# Autodesk Inventor assembly: SAR330
(part 2 of 2)
- to_ball3_2_Z@1 <-> to_rail_Z@57 [Mate]: SAR330-30_r:1 ↔ SAR3_ba:54
- to_ball3_2_YZ@1 <-> to_rail_YZ@57 [Angle] (0 deg): SAR330-30_r:1 ↔ SAR3_ba:54
- to_ball3_3_XY@1 <-> to_rail_XY@58 [Mate]: SAR330-30_r:1 ↔ SAR3_ba:55
- to_ball3_3_Z@1 <-> to_rail_Z@58 [Mate]: SAR330-30_r:1 ↔ SAR3_ba:55
- to_ball3_3_YZ@1 <-> to_rail_YZ@58 [Angle] (0 deg): SAR330-30_r:1 ↔ SAR3_ba:55
- to_ball3_4_XY@1 <-> to_rail_XY@59 [Mate]: SAR330-30_r:1 ↔ SAR3_ba:56
- to_ball3_4_Z@1 <-> to_rail_Z@59 [Mate]: SAR330-30_r:1 ↔ SAR3_ba:56
- to_ball3_4_YZ@1 <-> to_rail_YZ@59 [Angle] (0 deg): SAR330-30_r:1 ↔ SAR3_ba:56
- to_ball3_5_XY@1 <-> to_rail_XY@60 [Mate]: SAR330-30_r:1 ↔ SAR3_ba:57
- to_ball3_5_Z@1 <-> to_rail_Z@60 [Mate]: SAR330-30_r:1 ↔ SAR3_ba:57
- to_ball3_5_YZ@1 <-> to_rail_YZ@60 [Angle] (0 deg): SAR330-30_r:1 ↔ SAR3_ba:57
- to_ball3_6_XY@1 <-> to_rail_XY@61 [Mate]: SAR330-30_r:1 ↔ SAR3_ba:58
- to_ball3_6_Z@1 <-> to_rail_Z@61 [Mate]: SAR330-30_r:1 ↔ SAR3_ba:58
- to_ball3_6_YZ@1 <-> to_rail_YZ@61 [Angle] (0 deg): SAR330-30_r:1 ↔ SAR3_ba:58
- to_ball3_7_XY@1 <-> to_rail_XY@62 [Mate]: SAR330-30_r:1 ↔ SAR3_ba:59
- to_ball3_7_Z@1 <-> to_rail_Z@62 [Mate]: SAR330-30_r:1 ↔ SAR3_ba:59
- to_ball3_7_YZ@1 <-> to_rail_YZ@62 [Angle] (0 deg): SAR330-30_r:1 ↔ SAR3_ba:59
- to_ball3_8_XY@1 <-> to_rail_XY@63 [Mate]: SAR330-30_r:1 ↔ SAR3_ba:60
- to_ball3_8_Z@1 <-> to_rail_Z@63 [Mate]: SAR330-30_r:1 ↔ SAR3_ba:60
- to_ball3_8_YZ@1 <-> to_rail_YZ@63 [Angle] (0 deg): SAR330-30_r:1 ↔ SAR3_ba:60
- to_ball3_9_XY@1 <-> to_rail_XY@64 [Mate]: SAR330-30_r:1 ↔ SAR3_ba:61
- to_ball3_9_Z@1 <-> to_rail_Z@64 [Mate]: SAR330-30_r:1 ↔ SAR3_ba:61
- to_ball3_9_YZ@1 <-> to_rail_YZ@64 [Angle] (0 deg): SAR330-30_r:1 ↔ SAR3_ba:61
- to_ball3_10_XY@1 <-> to_rail_XY@65 [Mate]: SAR330-30_r:1 ↔ SAR3_ba:62
- to_ball3_10_Z@1 <-> to_rail_Z@65 [Mate]: SAR330-30_r:1 ↔ SAR3_ba:62
- to_ball3_10_YZ@1 <-> to_rail_YZ@65 [Angle] (0 deg): SAR330-30_r:1 ↔ SAR3_ba:62
- to_ball3_11_XY@1 <-> to_rail_XY@66 [Mate]: SAR330-30_r:1 ↔ SAR3_ba:63
- to_ball3_11_Z@1 <-> to_rail_Z@66 [Mate]: SAR330-30_r:1 ↔ SAR3_ba:63
- to_ball3_11_YZ@1 <-> to_rail_YZ@66 [Angle] (0 deg): SAR330-30_r:1 ↔ SAR3_ba:63
- to_ball3_12_XY@1 <-> to_rail_XY@67 [Mate]: SAR330-30_r:1 ↔ SAR3_ba:64
- to_ball3_12_Z@1 <-> to_rail_Z@67 [Mate]: SAR330-30_r:1 ↔ SAR3_ba:64
- to_ball3_12_YZ@1 <-> to_rail_YZ@67 [Angle] (0 deg): SAR330-30_r:1 ↔ SAR3_ba:64
- to_ball3_13_XY@1 <-> to_rail_XY@68 [Mate]: SAR330-30_r:1 ↔ SAR3_ba:65
- to_ball3_13_Z@1 <-> to_rail_Z@68 [Mate]: SAR330-30_r:1 ↔ SAR3_ba:65
- to_ball3_13_YZ@1 <-> to_rail_YZ@68 [Angle] (0 deg): SAR330-30_r:1 ↔ SAR3_ba:65
- to_ball3_14_XY@1 <-> to_rail_XY@69 [Mate]: SAR330-30_r:1 ↔ SAR3_ba:66
- to_ball3_14_Z@1 <-> to_rail_Z@69 [Mate]: SAR330-30_r:1 ↔ SAR3_ba:66
- to_ball3_14_YZ@1 <-> to_rail_YZ@69 [Angle] (0 deg): SAR330-30_r:1 ↔ SAR3_ba:66
- to_ball3_15_XY@1 <-> to_rail_XY@70 [Mate]: SAR330-30_r:1 ↔ SAR3_ba:67
- to_ball3_15_Z@1 <-> to_rail_Z@70 [Mate]: SAR330-30_r:1 ↔ SAR3_ba:67
- to_ball3_15_YZ@1 <-> to_rail_YZ@70 [Angle] (0 deg): SAR330-30_r:1 ↔ SAR3_ba:67
- to_ball3_16_XY@1 <-> to_rail_XY@71 [Mate]: SAR330-30_r:1 ↔ SAR3_ba:68
- to_ball3_16_Z@1 <-> to_rail_Z@71 [Mate]: SAR330-30_r:1 ↔ SAR3_ba:68
- to_ball3_16_YZ@1 <-> to_rail_YZ@71 [Angle] (0 deg): SAR330-30_r:1 ↔ SAR3_ba:68
- to_ball3_17_XY@1 <-> to_rail_XY@72 [Mate]: SAR330-30_r:1 ↔ SAR3_ba:69
- to_ball3_17_Z@1 <-> to_rail_Z@72 [Mate]: SAR330-30_r:1 ↔ SAR3_ba:69
- to_ball3_17_YZ@1 <-> to_rail_YZ@72 [Angle] (0 deg): SAR330-30_r:1 ↔ SAR3_ba:69
- to_ball3_18_XY@1 <-> to_rail_XY@73 [Mate]: SAR330-30_r:1 ↔ SAR3_ba:70
- to_ball3_18_Z@1 <-> to_rail_Z@73 [Mate]: SAR330-30_r:1 ↔ SAR3_ba:70
- to_ball3_18_YZ@1 <-> to_rail_YZ@73 [Angle] (0 deg): SAR330-30_r:1 ↔ SAR3_ba:70
- to_ball3_19_XY@1 <-> to_rail_XY@74 [Mate]: SAR330-30_r:1 ↔ SAR3_ba:71
- to_ball3_19_Z@1 <-> to_rail_Z@74 [Mate]: SAR330-30_r:1 ↔ SAR3_ba:71
- to_ball3_19_YZ@1 <-> to_rail_YZ@74 [Angle] (0 deg): SAR330-30_r:1 ↔ SAR3_ba:71
- to_ball3_20_XY@1 <-> to_rail_XY@75 [Mate]: SAR330-30_r:1 ↔ SAR3_ba:72
- to_ball3_20_Z@1 <-> to_rail_Z@75 [Mate]: SAR330-30_r:1 ↔ SAR3_ba:72
- to_ball3_20_YZ@1 <-> to_rail_YZ@75 [Angle] (0 deg): SAR330-30_r:1 ↔ SAR3_ba:72
- to_ball3_21_XY@1 <-> to_rail_XY@76 [Mate]: SAR330-30_r:1 ↔ SAR3_ba:73
- to_ball3_21_Z@1 <-> to_rail_Z@76 [Mate]: SAR330-30_r:1 ↔ SAR3_ba:73
- to_ball3_21_YZ@1 <-> to_rail_YZ@76 [Angle] (0 deg): SAR330-30_r:1 ↔ SAR3_ba:73
- to_ball3_22_XY@1 <-> to_rail_XY@77 [Mate]: SAR330-30_r:1 ↔ SAR3_ba:74
- to_ball3_22_Z@1 <-> to_rail_Z@77 [Mate]: SAR330-30_r:1 ↔ SAR3_ba:74
- to_ball3_22_YZ@1 <-> to_rail_YZ@77 [Angle] (0 deg): SAR330-30_r:1 ↔ SAR3_ba:74
- to_ball3_23_XY@1 <-> to_rail_XY@78 [Mate]: SAR330-30_r:1 ↔ SAR3_ba:75
- to_ball3_23_Z@1 <-> to_rail_Z@78 [Mate]: SAR330-30_r:1 ↔ SAR3_ba:75
- to_ball3_23_YZ@1 <-> to_rail_YZ@78 [Angle] (0 deg): SAR330-30_r:1 ↔ SAR3_ba:75
- to_ball3_24_XY@1 <-> to_rail_XY@79 [Mate]: SAR330-30_r:1 ↔ SAR3_ba:76
- to_ball3_24_Z@1 <-> to_rail_Z@79 [Mate]: SAR330-30_r:1 ↔ SAR3_ba:76
- to_ball3_24_YZ@1 <-> to_rail_YZ@79 [Angle] (0 deg): SAR330-30_r:1 ↔ SAR3_ba:76
- to_ball3_25_XY@1 <-> to_rail_XY@80 [Mate]: SAR330-30_r:1 ↔ SAR3_ba:77
- to_ball3_25_Z@1 <-> to_rail_Z@80 [Mate]: SAR330-30_r:1 ↔ SAR3_ba:77
- to_ball3_25_YZ@1 <-> to_rail_YZ@80 [Angle] (0 deg): SAR330-30_r:1 ↔ SAR3_ba:77
- to_ball3_26_XY@1 <-> to_rail_XY@81 [Mate]: SAR330-30_r:1 ↔ SAR3_ba:78
- to_ball3_26_Z@1 <-> to_rail_Z@81 [Mate]: SAR330-30_r:1 ↔ SAR3_ba:78
- to_ball3_26_YZ@1 <-> to_rail_YZ@81 [Angle] (0 deg): SAR330-30_r:1 ↔ SAR3_ba:78
- to_ball4_1_XY@1 <-> to_rail_XY@82 [Mate]: SAR330-30_r:1 ↔ SAR3_ba:79
- to_ball4_1_Z@1 <-> to_rail_Z@82 [Mate]: SAR330-30_r:1 ↔ SAR3_ba:79
- to_ball4_1_YZ@1 <-> to_rail_YZ@82 [Angle] (0 deg): SAR330-30_r:1 ↔ SAR3_ba:79
- to_ball4_2_XY@1 <-> to_rail_XY@83 [Mate]: SAR330-30_r:1 ↔ SAR3_ba:80
- to_ball4_2_Z@1 <-> to_rail_Z@83 [Mate]: SAR330-30_r:1 ↔ SAR3_ba:80
- to_ball4_2_YZ@1 <-> to_rail_YZ@83 [Angle] (0 deg): SAR330-30_r:1 ↔ SAR3_ba:80
- to_ball4_3_XY@1 <-> to_rail_XY@84 [Mate]: SAR330-30_r:1 ↔ SAR3_ba:81
- to_ball4_3_Z@1 <-> to_rail_Z@84 [Mate]: SAR330-30_r:1 ↔ SAR3_ba:81
- to_ball4_3_YZ@1 <-> to_rail_YZ@84 [Angle] (0 deg): SAR330-30_r:1 ↔ SAR3_ba:81
- to_ball4_4_XY@1 <-> to_rail_XY@85 [Mate]: SAR330-30_r:1 ↔ SAR3_ba:82
- to_ball4_4_Z@1 <-> to_rail_Z@85 [Mate]: SAR330-30_r:1 ↔ SAR3_ba:82
- to_ball4_4_YZ@1 <-> to_rail_YZ@85 [Angle] (0 deg): SAR330-30_r:1 ↔ SAR3_ba:82
- to_ball4_5_XY@1 <-> to_rail_XY@86 [Mate]: SAR330-30_r:1 ↔ SAR3_ba:83
- to_ball4_5_Z@1 <-> to_rail_Z@86 [Mate]: SAR330-30_r:1 ↔ SAR3_ba:83
- to_ball4_5_YZ@1 <-> to_rail_YZ@86 [Angle] (0 deg): SAR330-30_r:1 ↔ SAR3_ba:83
- to_ball4_6_XY@1 <-> to_rail_XY@87 [Mate]: SAR330-30_r:1 ↔ SAR3_ba:84
- to_ball4_6_Z@1 <-> to_rail_Z@87 [Mate]: SAR330-30_r:1 ↔ SAR3_ba:84
- to_ball4_6_YZ@1 <-> to_rail_YZ@87 [Angle] (0 deg): SAR330-30_r:1 ↔ SAR3_ba:84
- to_ball4_7_XY@1 <-> to_rail_XY@88 [Mate]: SAR330-30_r:1 ↔ SAR3_ba:85
- to_ball4_7_Z@1 <-> to_rail_Z@88 [Mate]: SAR330-30_r:1 ↔ SAR3_ba:85
- to_ball4_7_YZ@1 <-> to_rail_YZ@88 [Angle] (0 deg): SAR330-30_r:1 ↔ SAR3_ba:85
- to_ball4_8_XY@1 <-> to_rail_XY@89 [Mate]: SAR330-30_r:1 ↔ SAR3_ba:86
- to_ball4_8_Z@1 <-> to_rail_Z@89 [Mate]: SAR330-30_r:1 ↔ SAR3_ba:86
- to_ball4_8_YZ@1 <-> to_rail_YZ@89 [Angle] (0 deg): SAR330-30_r:1 ↔ SAR3_ba:86
- to_ball4_9_XY@1 <-> to_rail_XY@90 [Mate]: SAR330-30_r:1 ↔ SAR3_ba:87
- to_ball4_9_Z@1 <-> to_rail_Z@90 [Mate]: SAR330-30_r:1 ↔ SAR3_ba:87
- to_ball4_9_YZ@1 <-> to_rail_YZ@90 [Angle] (0 deg): SAR330-30_r:1 ↔ SAR3_ba:87
- to_ball4_10_XY@1 <-> to_rail_XY@91 [Mate]: SAR330-30_r:1 ↔ SAR3_ba:88
- to_ball4_10_Z@1 <-> to_rail_Z@91 [Mate]: SAR330-30_r:1 ↔ SAR3_ba:88
- to_ball4_10_YZ@1 <-> to_rail_YZ@91 [Angle] (0 deg): SAR330-30_r:1 ↔ SAR3_ba:88
- to_ball4_11_XY@1 <-> to_rail_XY@92 [Mate]: SAR330-30_r:1 ↔ SAR3_ba:89
- to_ball4_11_Z@1 <-> to_rail_Z@92 [Mate]: SAR330-30_r:1 ↔ SAR3_ba:89
- to_ball4_11_YZ@1 <-> to_rail_YZ@92 [Angle] (0 deg): SAR330-30_r:1 ↔ SAR3_ba:89
- to_ball4_12_XY@1 <-> to_rail_XY@93 [Mate]: SAR330-30_r:1 ↔ SAR3_ba:90
- to_ball4_12_Z@1 <-> to_rail_Z@93 [Mate]: SAR330-30_r:1 ↔ SAR3_ba:90
- to_ball4_12_YZ@1 <-> to_rail_YZ@93 [Angle] (0 deg): SAR330-30_r:1 ↔ SAR3_ba:90
- to_ball4_13_XY@1 <-> to_rail_XY@94 [Mate]: SAR330-30_r:1 ↔ SAR3_ba:91
- to_ball4_13_Z@1 <-> to_rail_Z@94 [Mate]: SAR330-30_r:1 ↔ SAR3_ba:91
- to_ball4_13_YZ@1 <-> to_rail_YZ@94 [Angle] (0 deg): SAR330-30_r:1 ↔ SAR3_ba:91
- to_ball4_14_XY@1 <-> to_rail_XY@95 [Mate]: SAR330-30_r:1 ↔ SAR3_ba:92
- to_ball4_14_Z@1 <-> to_rail_Z@95 [Mate]: SAR330-30_r:1 ↔ SAR3_ba:92
- to_ball4_14_YZ@1 <-> to_rail_YZ@95 [Angle] (0 deg): SAR330-30_r:1 ↔ SAR3_ba:92
- to_ball4_15_XY@1 <-> to_rail_XY@96 [Mate]: SAR330-30_r:1 ↔ SAR3_ba:93
- to_ball4_15_Z@1 <-> to_rail_Z@96 [Mate]: SAR330-30_r:1 ↔ SAR3_ba:93
- to_ball4_15_YZ@1 <-> to_rail_YZ@96 [Angle] (0 deg): SAR330-30_r:1 ↔ SAR3_ba:93
- to_ball4_16_XY@1 <-> to_rail_XY@97 [Mate]: SAR330-30_r:1 ↔ SAR3_ba:94
- to_ball4_16_Z@1 <-> to_rail_Z@97 [Mate]: SAR330-30_r:1 ↔ SAR3_ba:94
- to_ball4_16_YZ@1 <-> to_rail_YZ@97 [Angle] (0 deg): SAR330-30_r:1 ↔ SAR3_ba:94
- to_ball4_17_XY@1 <-> to_rail_XY@98 [Mate]: SAR330-30_r:1 ↔ SAR3_ba:95
- to_ball4_17_Z@1 <-> to_rail_Z@98 [Mate]: SAR330-30_r:1 ↔ SAR3_ba:95
- to_ball4_17_YZ@1 <-> to_rail_YZ@98 [Angle] (0 deg): SAR330-30_r:1 ↔ SAR3_ba:95
- to_ball4_18_XY@1 <-> to_rail_XY@99 [Mate]: SAR330-30_r:1 ↔ SAR3_ba:96
- to_ball4_18_Z@1 <-> to_rail_Z@99 [Mate]: SAR330-30_r:1 ↔ SAR3_ba:96
- to_ball4_18_YZ@1 <-> to_rail_YZ@99 [Angle] (0 deg): SAR330-30_r:1 ↔ SAR3_ba:96
- to_ball4_19_XY@1 <-> to_rail_XY@100 [Mate]: SAR330-30_r:1 ↔ SAR3_ba:97
- to_ball4_19_Z@1 <-> to_rail_Z@100 [Mate]: SAR330-30_r:1 ↔ SAR3_ba:97
- to_ball4_19_YZ@1 <-> to_rail_YZ@100 [Angle] (0 deg): SAR330-30_r:1 ↔ SAR3_ba:97
- to_ball4_20_XY@1 <-> to_rail_XY@101 [Mate]: SAR330-30_r:1 ↔ SAR3_ba:98
- to_ball4_20_Z@1 <-> to_rail_Z@101 [Mate]: SAR330-30_r:1 ↔ SAR3_ba:98
- to_ball4_20_YZ@1 <-> to_rail_YZ@101 [Angle] (0 deg): SAR330-30_r:1 ↔ SAR3_ba:98
- to_ball4_21_XY@1 <-> to_rail_XY@102 [Mate]: SAR330-30_r:1 ↔ SAR3_ba:99
- to_ball4_21_Z@1 <-> to_rail_Z@102 [Mate]: SAR330-30_r:1 ↔ SAR3_ba:99
- to_ball4_21_YZ@1 <-> to_rail_YZ@102 [Angle] (0 deg): SAR330-30_r:1 ↔ SAR3_ba:99
- to_ball4_22_XY@1 <-> to_rail_XY@103 [Mate]: SAR330-30_r:1 ↔ SAR3_ba:100
- to_ball4_22_Z@1 <-> to_rail_Z@103 [Mate]: SAR330-30_r:1 ↔ SAR3_ba:100
- to_ball4_22_YZ@1 <-> to_rail_YZ@103 [Angle] (0 deg): SAR330-30_r:1 ↔ SAR3_ba:100
- to_ball4_23_XY@1 <-> to_rail_XY@104 [Mate]: SAR330-30_r:1 ↔ SAR3_ba:101
- to_ball4_23_Z@1 <-> to_rail_Z@104 [Mate]: SAR330-30_r:1 ↔ SAR3_ba:101
- to_ball4_23_YZ@1 <-> to_rail_YZ@104 [Angle] (0 deg): SAR330-30_r:1 ↔ SAR3_ba:101
- to_ball4_24_XY@1 <-> to_rail_XY@105 [Mate]: SAR330-30_r:1 ↔ SAR3_ba:102
- to_ball4_24_Z@1 <-> to_rail_Z@105 [Mate]: SAR330-30_r:1 ↔ SAR3_ba:102
- to_ball4_24_YZ@1 <-> to_rail_YZ@105 [Angle] (0 deg): SAR330-30_r:1 ↔ SAR3_ba:102
- to_ball4_25_XY@1 <-> to_rail_XY@106 [Mate]: SAR330-30_r:1 ↔ SAR3_ba:103
- to_ball4_25_Z@1 <-> to_rail_Z@106 [Mate]: SAR330-30_r:1 ↔ SAR3_ba:103
- to_ball4_25_YZ@1 <-> to_rail_YZ@106 [Angle] (0 deg): SAR330-30_r:1 ↔ SAR3_ba:103
- to_ball4_26_XY@1 <-> to_rail_XY@107 [Mate]: SAR330-30_r:1 ↔ SAR3_ba:104
- to_ball4_26_Z@1 <-> to_rail_Z@107 [Mate]: SAR330-30_r:1 ↔ SAR3_ba:104
- to_ball4_26_YZ@1 <-> to_rail_YZ@107 [Angle] (0 deg): SAR330-30_r:1 ↔ SAR3_ba:104
